# Autodesk Inventor assembly: Основная сборка
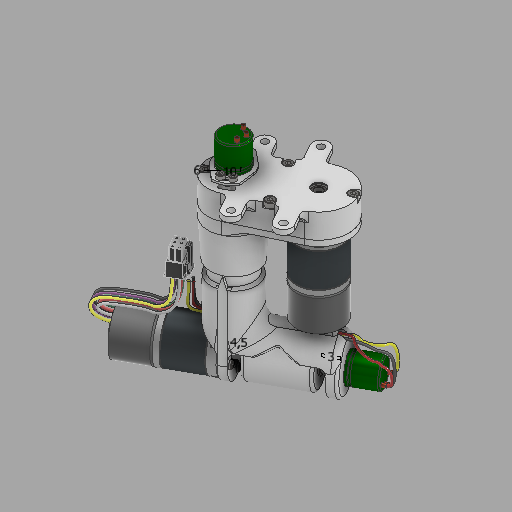
[picture p0: Inventor's stored thumbnail of the model, 512x512]
Saved by Autodesk Inventor 2025 (Build 290162000, 162)
## iProperties
Created: 2025-04-08
Part Number: Основная сборка
Document SubType Name: Assembly
Designer: Artem Sannikov
Author: Artem Sannikov
## Documents named in this file (27)
- C:\Users\Artem Sannikov\Desktop\Two_axis_gimbal\3D_модели\Основная сборка\Основная сборка.iam
- C:\Users\Artem Sannikov\Desktop\Two_axis_gimbal\3D_модели\Основная сборка\BLDC_3626.ipt
- C:\Users\Artem Sannikov\Desktop\Two_axis_gimbal\3D_модели\Основная сборка\GT2 40T 8 Bore v2.iam
- C:\Users\Artem Sannikov\Desktop\Two_axis_gimbal\3D_модели\Основная сборка\Энкодер P3022-V1-CW360.ipt
- C:\Users\Artem Sannikov\Desktop\Two_axis_gimbal\3D_модели\Основная сборка\Ремень.ipt
- C:\Users\Artem Sannikov\Desktop\Two_axis_gimbal\3D_модели\Основная сборка\Pulley_2.ipt
- C:\Users\Artem Sannikov\Desktop\Two_axis_gimbal\3D_модели\Основная сборка\Вал вертикальной оси.ipt
- C:\Users\Artem Sannikov\Desktop\Two_axis_gimbal\3D_модели\Основная сборка\Основная сборка\Мастер проектирования\Подшипник2.iam
- C:\Users\Artem Sannikov\Desktop\Two_axis_gimbal\3D_модели\Основная сборка\Основная сборка\Мастер проектирования\Подшипник5.iam
- C:\Users\Artem Sannikov\Desktop\Two_axis_gimbal\3D_модели\Основная сборка\Крпеление 2 оси.ipt
- C:\Users\Artem Sannikov\Desktop\Two_axis_gimbal\3D_модели\Основная сборка\Нижняя половина редуктора.ipt
- C:\Users\Artem Sannikov\Desktop\Two_axis_gimbal\3D_модели\Основная сборка\Вал 2 оси.ipt
- C:\Users\Artem Sannikov\Desktop\Two_axis_gimbal\3D_модели\Основная сборка\Крпеление ОУ.ipt
- C:\Users\Artem Sannikov\Documents\Inventor\Content Center Files\R2025\ru-RU\ISO 7380-1\ISO 7380-1 - M4 x 16.ipt
- C:\Users\Artem Sannikov\Documents\Inventor\Content Center Files\R2025\ru-RU\DIN 912\DIN 912 - M2 x 0,4 x 10 x 9.ipt
- C:\Users\Artem Sannikov\Documents\Inventor\Content Center Files\R2025\ru-RU\GOST 23360-78 (1)\Шпонка 4x4x8 ГОСТ 23360-78.ipt
- C:\Users\Artem Sannikov\Documents\Inventor\Content Center Files\R2025\ru-RU\GOST 13942-86 10mm _= 165mm\Кольцо A12 ГОСТ 13942-86.ipt
- C:\Users\Artem Sannikov\Documents\Inventor\Content Center Files\R2025\ru-RU\DIN 916\DIN 916 - M3  x  4.ipt
- C:\Users\Artem Sannikov\Documents\Inventor\Content Center Files\R2025\ru-RU\GOST 23360-78 (1)\Шпонка 4x4x40 ГОСТ 23360-78.ipt
- C:\Users\Artem Sannikov\Desktop\Two_axis_gimbal\3D_модели\Основная сборка\Фланец.ipt
- C:\Users\Artem Sannikov\Documents\Inventor\Content Center Files\R2025\ru-RU\DIN 912\DIN 912 - M2 x 0,4 x 4 x 3.ipt
- C:\Users\Artem Sannikov\Desktop\Two_axis_gimbal\3D_модели\Основная сборка\Верх редуктора.ipt
- C:\Users\Artem Sannikov\Documents\Inventor\Content Center Files\R2025\ru-RU\DIN 912\DIN 912 - M3 x 0,5 x 10 x 8,75.ipt
- C:\Users\Artem Sannikov\Documents\Inventor\Content Center Files\R2025\ru-RU\DIN 912\DIN 912 - M4 x 0,7 x 20 x 18,25.ipt
- C:\Users\Artem Sannikov\Documents\Inventor\Content Center Files\R2025\ru-RU\DIN 912\DIN 912 - M3 x 0,5 x 8 x 6,75.ipt
- C:\Users\Artem Sannikov\Desktop\Two_axis_gimbal\3D_модели\Провода.ipt
- C:\Users\Artem Sannikov\Desktop\Two_axis_gimbal\3D_модели\Основная сборка\ATX-12V-6-Pin.iam
## Components (53 placed, 25 different names)
1. BLDC_3626:1 — Совмещение:1, Заподлицо:1, Заподлицо:3, Совмещение:8, Совмещение:15, Заподлицо:10
2. GT2 40T 8 Bore v2:1 [sub-assembly] — Совмещение:1, Заподлицо:5, Совмещение:8, Совмещение:31
3. Энкодер P3022-V1-CW360:1 — Совмещение:9, Совмещение:10, Совмещение:12, Заподлицо:6, Заподлицо:15
4. Ремень:1 — Заподлицо:5, Совмещение:9, Совмещение:11
5. Pulley_2:1 — Совмещение:10, Совмещение:11, Совмещение:12, Заподлицо:7, Заподлицо:8, Заподлицо:12
6. Вал вертикальной оси:1 — Заподлицо:6, Заподлицо:7, Заподлицо:8, Совмещение:13, Совмещение:14, Заподлицо:9, Совмещение:23, Совмещение:24, Совмещение:25, Заподлицо:12, Совмещение:29, Совмещение:30, Совмещение:39, Касательность:3
7. Подшипник:1 [sub-assembly] — Совмещение:13, Совмещение:22
8. Подшипник:2 [sub-assembly] — Совмещение:14, Совмещение:30, Заподлицо:16
9. Подшипник:3 [sub-assembly] — Совмещение:15, Совмещение:31
10. Крпеление 2 оси:1 — Заподлицо:9, Совмещение:17, Совмещение:19, Вставка:1, Вставка:2, Вставка:3, Вставка:4, Вставка:5, Вставка:6, Вставка:19, Вставка:20, Вставка:21, Вставка:22, Заподлицо:17
11. BLDC_3626:2 — Совмещение:17, Совмещение:18, Заподлицо:11
12. Нижняя половина редуктора:1 — Заподлицо:10, Совмещение:22, Вставка:23, Вставка:24, Вставка:25, Вставка:26, Заподлицо:17
13. Энкодер P3022-V1-CW360:2 — Совмещение:18, Совмещение:19, Заподлицо:18, Заподлицо:19, Заподлицо:20
14. Вал 2 оси:1 — Заподлицо:11, Совмещение:21, Совмещение:26, Совмещение:27, Заподлицо:13, Совмещение:32, Совмещение:33, Совмещение:34, Совмещение:35, Касательность:1, Касательность:2, Заподлицо:14, Совмещение:36, Совмещение:37, Совмещение:38
15. Крпеление ОУ:1 — Совмещение:21, Совмещение:28, Заподлицо:13, Заподлицо:14
16. ISO 7380-1 M4 x 16:1 — Вставка:1
17. ISO 7380-1 M4 x 16:2 — Вставка:2
18. DIN 912 - заменено на DIN EN ISO 4762 M2 x 10:1 — Вставка:3
19. DIN 912 - заменено на DIN EN ISO 4762 M2 x 10:2 — Вставка:4
20. DIN 912 - заменено на DIN EN ISO 4762 M2 x 10:3 — Вставка:5
21. DIN 912 - заменено на DIN EN ISO 4762 M2 x 10:4 — Вставка:6
22. Шпонка ГОСТ 23360-78 4 x 4 x 8:1 — Совмещение:23, Совмещение:24, Совмещение:25
23. Кольцо A ГОСТ 13942-86 12:1 — Совмещение:26, Совмещение:27, Совмещение:28
24. Кольцо A ГОСТ 13942-86 12:2 — Совмещение:29
25. Кольцо A ГОСТ 13942-86 12:3 — Совмещение:32, Совмещение:33
26. DIN 916 M3  x  4:2 — Совмещение:34, Касательность:1
27. DIN 916 M3  x  4:3 — Совмещение:35, Касательность:2
28. DIN 916 M3  x  4:5 — Совмещение:39, Касательность:3
29. Шпонка ГОСТ 23360-78 4 x 4 x 40:1 — Совмещение:36, Совмещение:37, Совмещение:38
30. Фланец:1 — Заподлицо:15, Вставка:7, Вставка:8, Вставка:9, Вставка:10, Вставка:11, Вставка:12, Вставка:13, Вставка:14
31. DIN 912 - заменено на DIN EN ISO 4762 M2 x 4:1 — Вставка:7
32. DIN 912 - заменено на DIN EN ISO 4762 M2 x 4:2 — Вставка:8
33. DIN 912 - заменено на DIN EN ISO 4762 M2 x 4:3 — Вставка:9
34. DIN 912 - заменено на DIN EN ISO 4762 M2 x 4:4 — Вставка:10
35. Верх редуктора:1 — Заподлицо:16, Вставка:15, Вставка:16, Вставка:17, Вставка:18
36. DIN 912 - заменено на DIN EN ISO 4762 M3 x 10:1 — Вставка:11
37. DIN 912 - заменено на DIN EN ISO 4762 M3 x 10:2 — Вставка:12
38. DIN 912 - заменено на DIN EN ISO 4762 M3 x 10:3 — Вставка:13
39. DIN 912 - заменено на DIN EN ISO 4762 M3 x 10:4 — Вставка:14
40. DIN 912 - заменено на DIN EN ISO 4762 M4 x 20:1 — Вставка:15
41. DIN 912 - заменено на DIN EN ISO 4762 M4 x 20:2 — Вставка:16
42. DIN 912 - заменено на DIN EN ISO 4762 M4 x 20:3 — Вставка:17
43. DIN 912 - заменено на DIN EN ISO 4762 M4 x 20:4 — Вставка:18
44. DIN 912 - заменено на DIN EN ISO 4762 M3 x 8:1 — Вставка:19
45. DIN 912 - заменено на DIN EN ISO 4762 M3 x 8:2 — Вставка:20
46. DIN 912 - заменено на DIN EN ISO 4762 M3 x 8:3 — Вставка:21
47. DIN 912 - заменено на DIN EN ISO 4762 M3 x 8:4 — Вставка:22
48. DIN 912 - заменено на DIN EN ISO 4762 M3 x 8:5 — Вставка:23
49. DIN 912 - заменено на DIN EN ISO 4762 M3 x 8:6 — Вставка:24
50. DIN 912 - заменено на DIN EN ISO 4762 M3 x 8:7 — Вставка:25
51. DIN 912 - заменено на DIN EN ISO 4762 M3 x 8:8 — Вставка:26
52. Провода:1 — Заподлицо:18, Заподлицо:19, Заподлицо:20
53. ATX-12V-6-Pin:1 [sub-assembly]
## Relationships (81: Mate 33, Insert 26, Flush 19, Tangent 3)
- Совмещение:1 [Mate]: BLDC_3626:1 ↔ GT2 40T 8 Bore v2:1
- Заподлицо:1 [Flush]: BLDC_3626:1
- Заподлицо:2 [Flush] (-50 mm)
- Совмещение:3 [Mate]
- Совмещение:4 [Mate]
- Заподлицо:3 [Flush]: BLDC_3626:1
- Заподлицо:5 [Flush]: GT2 40T 8 Bore v2:1 ↔ Ремень:1
- Совмещение:8 [Mate]: BLDC_3626:1 ↔ GT2 40T 8 Bore v2:1
- Совмещение:9 [Mate]: Энкодер P3022-V1-CW360:1 ↔ Ремень:1
- Совмещение:10 [Mate]: Энкодер P3022-V1-CW360:1 ↔ Pulley_2:1
- Совмещение:11 [Mate]: Ремень:1 ↔ Pulley_2:1
- Совмещение:12 [Mate] (10 mm): Энкодер P3022-V1-CW360:1 ↔ Pulley_2:1
- Заподлицо:6 [Flush]: Энкодер P3022-V1-CW360:1 ↔ Вал вертикальной оси:1
- Заподлицо:7 [Flush]: Pulley_2:1 ↔ Вал вертикальной оси:1
- Заподлицо:8 [Flush]: Pulley_2:1 ↔ Вал вертикальной оси:1
- Совмещение:13 [Mate]: Вал вертикальной оси:1 ↔ Подшипник:1
- Совмещение:14 [Mate]: Вал вертикальной оси:1 ↔ Подшипник:2
- Совмещение:15 [Mate]: BLDC_3626:1 ↔ Подшипник:3
- Заподлицо:9 [Flush]: Вал вертикальной оси:1 ↔ Крпеление 2 оси:1
- Совмещение:17 [Mate]: Крпеление 2 оси:1 ↔ BLDC_3626:2
- Заподлицо:10 [Flush]: BLDC_3626:1 ↔ Нижняя половина редуктора:1
- Совмещение:18 [Mate]: BLDC_3626:2 ↔ Энкодер P3022-V1-CW360:2
- Совмещение:19 [Mate]: Крпеление 2 оси:1 ↔ Энкодер P3022-V1-CW360:2
- Заподлицо:11 [Flush]: BLDC_3626:2 ↔ Вал 2 оси:1
- Совмещение:21 [Mate]: Вал 2 оси:1 ↔ Крпеление ОУ:1
- Совмещение:22 [Mate]: Подшипник:1 ↔ Нижняя половина редуктора:1
- Вставка:1 [Insert]: Крпеление 2 оси:1 ↔ ISO 7380-1 M4 x 16:1
- Вставка:2 [Insert]: Крпеление 2 оси:1 ↔ ISO 7380-1 M4 x 16:2
- Вставка:3 [Insert]: Крпеление 2 оси:1 ↔ DIN 912 - заменено на DIN EN ISO 4762 M2 x 10:1
- Вставка:4 [Insert]: Крпеление 2 оси:1 ↔ DIN 912 - заменено на DIN EN ISO 4762 M2 x 10:2
- Вставка:5 [Insert]: Крпеление 2 оси:1 ↔ DIN 912 - заменено на DIN EN ISO 4762 M2 x 10:3
- Вставка:6 [Insert]: Крпеление 2 оси:1 ↔ DIN 912 - заменено на DIN EN ISO 4762 M2 x 10:4
- Совмещение:23 [Mate]: Вал вертикальной оси:1 ↔ Шпонка ГОСТ 23360-78 4 x 4 x 8:1
- Совмещение:24 [Mate]: Вал вертикальной оси:1 ↔ Шпонка ГОСТ 23360-78 4 x 4 x 8:1
- Совмещение:25 [Mate]: Вал вертикальной оси:1 ↔ Шпонка ГОСТ 23360-78 4 x 4 x 8:1
- Совмещение:26 [Mate]: Вал 2 оси:1 ↔ Кольцо A ГОСТ 13942-86 12:1
- Совмещение:27 [Mate]: Вал 2 оси:1 ↔ Кольцо A ГОСТ 13942-86 12:1
- Совмещение:28 [Mate]: Крпеление ОУ:1 ↔ Кольцо A ГОСТ 13942-86 12:1
- Заподлицо:12 [Flush]: Pulley_2:1 ↔ Вал вертикальной оси:1
- Совмещение:29 [Mate]: Вал вертикальной оси:1 ↔ Кольцо A ГОСТ 13942-86 12:2
- Совмещение:30 [Mate]: Вал вертикальной оси:1 ↔ Подшипник:2
- Совмещение:31 [Mate] (1 mm): GT2 40T 8 Bore v2:1 ↔ Подшипник:3
- Заподлицо:13 [Flush]: Вал 2 оси:1 ↔ Крпеление ОУ:1
- Совмещение:32 [Mate]: Вал 2 оси:1 ↔ Кольцо A ГОСТ 13942-86 12:3
- Совмещение:33 [Mate]: Вал 2 оси:1 ↔ Кольцо A ГОСТ 13942-86 12:3
- Совмещение:34 [Mate]: Вал 2 оси:1 ↔ DIN 916 M3  x  4:2
- Совмещение:35 [Mate]: Вал 2 оси:1 ↔ DIN 916 M3  x  4:3
- Касательность:1 [Tangent]: Вал 2 оси:1 ↔ DIN 916 M3  x  4:2
- Касательность:2 [Tangent]: Вал 2 оси:1 ↔ DIN 916 M3  x  4:3
- Заподлицо:14 [Flush]: Вал 2 оси:1 ↔ Крпеление ОУ:1
- Совмещение:36 [Mate]: Вал 2 оси:1 ↔ Шпонка ГОСТ 23360-78 4 x 4 x 40:1
- Совмещение:37 [Mate]: Вал 2 оси:1 ↔ Шпонка ГОСТ 23360-78 4 x 4 x 40:1
- Совмещение:38 [Mate]: Вал 2 оси:1 ↔ Шпонка ГОСТ 23360-78 4 x 4 x 40:1
- Совмещение:39 [Mate]: Вал вертикальной оси:1 ↔ DIN 916 M3  x  4:5
- Касательность:3 [Tangent]: Вал вертикальной оси:1 ↔ DIN 916 M3  x  4:5
- Заподлицо:15 [Flush]: Энкодер P3022-V1-CW360:1 ↔ Фланец:1
- Вставка:7 [Insert]: Фланец:1 ↔ DIN 912 - заменено на DIN EN ISO 4762 M2 x 4:1
- Вставка:8 [Insert]: Фланец:1 ↔ DIN 912 - заменено на DIN EN ISO 4762 M2 x 4:2
- Вставка:9 [Insert]: Фланец:1 ↔ DIN 912 - заменено на DIN EN ISO 4762 M2 x 4:3
- Вставка:10 [Insert]: Фланец:1 ↔ DIN 912 - заменено на DIN EN ISO 4762 M2 x 4:4
- Заподлицо:16 [Flush]: Подшипник:2 ↔ Верх редуктора:1
- Вставка:11 [Insert]: Фланец:1 ↔ DIN 912 - заменено на DIN EN ISO 4762 M3 x 10:1
- Вставка:12 [Insert]: Фланец:1 ↔ DIN 912 - заменено на DIN EN ISO 4762 M3 x 10:2
- Вставка:13 [Insert]: Фланец:1 ↔ DIN 912 - заменено на DIN EN ISO 4762 M3 x 10:3
- Вставка:14 [Insert]: Фланец:1 ↔ DIN 912 - заменено на DIN EN ISO 4762 M3 x 10:4
- Вставка:15 [Insert]: Верх редуктора:1 ↔ DIN 912 - заменено на DIN EN ISO 4762 M4 x 20:1
- Вставка:16 [Insert]: Верх редуктора:1 ↔ DIN 912 - заменено на DIN EN ISO 4762 M4 x 20:2
- Вставка:17 [Insert]: Верх редуктора:1 ↔ DIN 912 - заменено на DIN EN ISO 4762 M4 x 20:3
- Вставка:18 [Insert]: Верх редуктора:1 ↔ DIN 912 - заменено на DIN EN ISO 4762 M4 x 20:4
- Вставка:19 [Insert]: Крпеление 2 оси:1 ↔ DIN 912 - заменено на DIN EN ISO 4762 M3 x 8:1
- Вставка:20 [Insert]: Крпеление 2 оси:1 ↔ DIN 912 - заменено на DIN EN ISO 4762 M3 x 8:2
- Вставка:21 [Insert]: Крпеление 2 оси:1 ↔ DIN 912 - заменено на DIN EN ISO 4762 M3 x 8:3
- Вставка:22 [Insert]: Крпеление 2 оси:1 ↔ DIN 912 - заменено на DIN EN ISO 4762 M3 x 8:4
- Вставка:23 [Insert]: Нижняя половина редуктора:1 ↔ DIN 912 - заменено на DIN EN ISO 4762 M3 x 8:5
- Вставка:24 [Insert]: Нижняя половина редуктора:1 ↔ DIN 912 - заменено на DIN EN ISO 4762 M3 x 8:6
- Вставка:25 [Insert]: Нижняя половина редуктора:1 ↔ DIN 912 - заменено на DIN EN ISO 4762 M3 x 8:7
- Вставка:26 [Insert]: Нижняя половина редуктора:1 ↔ DIN 912 - заменено на DIN EN ISO 4762 M3 x 8:8
- Заподлицо:17 [Flush]: Крпеление 2 оси:1 ↔ Нижняя половина редуктора:1
- Заподлицо:18 [Flush]: Энкодер P3022-V1-CW360:2 ↔ Провода:1
- Заподлицо:19 [Flush]: Энкодер P3022-V1-CW360:2 ↔ Провода:1
- Заподлицо:20 [Flush]: Энкодер P3022-V1-CW360:2 ↔ Провода:1
